# Autodesk Inventor assembly: UpperBody
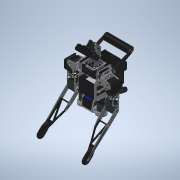
[picture p0: Inventor's stored thumbnail of the model, 180x180]
Saved by Autodesk Inventor 2020.4 (Build 244396000, 396)
## iProperties
Created: 2016-05-03
Part Number: UpperBody
Document SubType Name: Assembly
Designer: hiroaki
Mass: 2419.66 g
Surface Area: 8002.44 cm^2
Volume: 1435.02 cm^3
Density: 1.68615 g/cm^3
Author: hiroaki
## Documents named in this file (9)
- C:\Users\Masato\Documents\Inventor\CIT Brains_Inventor\OpenPlatform_ver3_0\UpperBody.iam
- C:\Users\Masato\Documents\Inventor\CIT Brains_Inventor\OpenPlatform_ver3_0\UpperBody\Trunk\Trunk.iam
- C:\Users\Masato\Documents\Inventor\CIT Brains_Inventor\OpenPlatform_ver3_0\UpperBody\Head\Head.iam
- C:\Users\Masato\Documents\Inventor\CIT Brains_Inventor\OpenPlatform_ver3_0\UpperBody\Arm\ForeArm.iam
- C:\Users\Masato\Documents\Inventor\CIT Brains_Inventor\OpenPlatform_ver3_0\UpperBody\Arm\Shoulder.iam
- C:\Users\Masato\Documents\Inventor\CIT Brains_Inventor\OpenPlatform_ver3_0\UpperBody\Arm\UpperArm.iam
- C:\Users\Masato\Documents\Inventor\CIT Brains_Inventor\OpenPlatform_ver3_0\UpperBody\Arm\SideBumper.ipt
- C:\Users\Masato\Documents\Inventor\CIT Brains_Inventor\OpenPlatform_ver3_0\Ready_Made\Screw\M2_6-6.ipt
- C:\Users\Masato\Documents\Inventor\CIT Brains_Inventor\OpenPlatform_ver3_0\Ready_Made\Screw\M2_6-8.ipt
## Components (54 placed, 8 different names)
1. Head:1 [sub-assembly] — 挿入:13, 角度:12, 挿入:82, 挿入:83, 挿入:84, 挿入:85
2. Trunk:1 [sub-assembly] — 挿入:13, 角度:12, 挿入:22, 挿入:23, 角度:22
3. ForeArm:1 [sub-assembly] — 角度:18, 挿入:21, 角度:19, 挿入:66, 挿入:67, 挿入:68, 挿入:69, 挿入:70, 挿入:71, 挿入:72, 挿入:73
4. UpperArm:1 [sub-assembly] — 挿入:21, 角度:19, メイト:4, 角度:20, メイト:5, 挿入:25
5. ForeArm:2 [sub-assembly] — 挿入:19, 角度:18, 挿入:74, 挿入:75, 挿入:76, 挿入:77, 挿入:78, 挿入:79, 挿入:80, 挿入:81
6. UpperArm:2 [sub-assembly] — 挿入:19, メイト:3, 角度:21, メイト:6, 挿入:24
7. SideBumper:1 — メイト:4, 角度:20, メイト:5
8. SideBumper:2 — メイト:3, 角度:21, メイト:6
9. Shoulder:1 [sub-assembly] — 挿入:22, 挿入:25, 角度:22, 角度:23, 挿入:42, 挿入:43, 挿入:44, 挿入:45, 挿入:46, 挿入:47, 挿入:48, 挿入:49, 挿入:50, 挿入:51, 挿入:52, 挿入:53
10. Shoulder:2 [sub-assembly] — 挿入:23, 挿入:24, 角度:23, 挿入:54, 挿入:55, 挿入:56, 挿入:57, 挿入:58, 挿入:59, 挿入:60, 挿入:61, 挿入:62, 挿入:63, 挿入:64, 挿入:65
11. M2_6-6:1 — 挿入:42
12. M2_6-6:2 — 挿入:43
13. M2_6-6:3 — 挿入:44
14. M2_6-6:4 — 挿入:45
15. M2_6-6:5 — 挿入:46
16. M2_6-6:6 — 挿入:47
17. M2_6-6:7 — 挿入:48
18. M2_6-6:8 — 挿入:49
19. M2_6-6:9 — 挿入:50
20. M2_6-6:10 — 挿入:51
21. M2_6-6:11 — 挿入:52
22. M2_6-6:12 — 挿入:53
23. M2_6-6:13 — 挿入:54
24. M2_6-6:14 — 挿入:55
25. M2_6-6:15 — 挿入:56
26. M2_6-6:16 — 挿入:57
27. M2_6-6:17 — 挿入:58
28. M2_6-6:18 — 挿入:59
29. M2_6-6:19 — 挿入:60
30. M2_6-6:20 — 挿入:61
31. M2_6-6:21 — 挿入:62
32. M2_6-6:22 — 挿入:63
33. M2_6-6:23 — 挿入:64
34. M2_6-6:24 — 挿入:65
35. M2_6-6:25 — 挿入:66
36. M2_6-6:26 — 挿入:67
37. M2_6-6:27 — 挿入:68
38. M2_6-6:28 — 挿入:69
39. M2_6-6:29 — 挿入:70
40. M2_6-6:30 — 挿入:71
41. M2_6-6:31 — 挿入:72
42. M2_6-6:32 — 挿入:73
43. M2_6-6:33 — 挿入:74
44. M2_6-6:34 — 挿入:75
45. M2_6-6:35 — 挿入:76
46. M2_6-6:36 — 挿入:77
47. M2_6-6:37 — 挿入:78
48. M2_6-6:38 — 挿入:79
49. M2_6-6:39 — 挿入:81
50. M2_6-6:40 — 挿入:80
51. M2_6-8:1 — 挿入:82
52. M2_6-8:2 — 挿入:83
53. M2_6-8:3 — 挿入:84
54. M2_6-8:4 — 挿入:85
## Relationships (62: Insert 51, Angle 7, Mate 4)
- 挿入:13 [Insert]: Head:1 ↔ Trunk:1
- 角度:12 [Angle] (0 deg): Head:1 ↔ Trunk:1
- 挿入:19 [Insert]: ForeArm:2 ↔ UpperArm:2
- 角度:18 [Angle] (0 deg): ForeArm:1 ↔ ForeArm:2
- 挿入:21 [Insert]: ForeArm:1 ↔ UpperArm:1
- 角度:19 [Angle] (45 deg): ForeArm:1 ↔ UpperArm:1
- メイト:3 [Mate]: UpperArm:2 ↔ SideBumper:2
- メイト:4 [Mate]: UpperArm:1 ↔ SideBumper:1
- 角度:20 [Angle] (0 deg): UpperArm:1 ↔ SideBumper:1
- メイト:5 [Mate]: UpperArm:1 ↔ SideBumper:1
- 角度:21 [Angle] (0 deg): UpperArm:2 ↔ SideBumper:2
- メイト:6 [Mate]: UpperArm:2 ↔ SideBumper:2
- 挿入:22 [Insert]: Trunk:1 ↔ Shoulder:1
- 挿入:23 [Insert]: Trunk:1 ↔ Shoulder:2
- 挿入:24 [Insert]: UpperArm:2 ↔ Shoulder:2
- 挿入:25 [Insert]: UpperArm:1 ↔ Shoulder:1
- 角度:22 [Angle] (0 deg): Trunk:1 ↔ Shoulder:1
- 角度:23 [Angle] (0 deg): Shoulder:1 ↔ Shoulder:2
- 挿入:42 [Insert]: Shoulder:1 ↔ M2_6-6:1
- 挿入:43 [Insert]: Shoulder:1 ↔ M2_6-6:2
- 挿入:44 [Insert]: Shoulder:1 ↔ M2_6-6:3
- 挿入:45 [Insert]: Shoulder:1 ↔ M2_6-6:4
- 挿入:46 [Insert]: Shoulder:1 ↔ M2_6-6:5
- 挿入:47 [Insert]: Shoulder:1 ↔ M2_6-6:6
- 挿入:48 [Insert]: Shoulder:1 ↔ M2_6-6:7
- 挿入:49 [Insert]: Shoulder:1 ↔ M2_6-6:8
- 挿入:50 [Insert]: Shoulder:1 ↔ M2_6-6:9
- 挿入:51 [Insert]: Shoulder:1 ↔ M2_6-6:10
- 挿入:52 [Insert]: Shoulder:1 ↔ M2_6-6:11
- 挿入:53 [Insert]: Shoulder:1 ↔ M2_6-6:12
- 挿入:54 [Insert]: Shoulder:2 ↔ M2_6-6:13
- 挿入:55 [Insert]: Shoulder:2 ↔ M2_6-6:14
- 挿入:56 [Insert]: Shoulder:2 ↔ M2_6-6:15
- 挿入:57 [Insert]: Shoulder:2 ↔ M2_6-6:16
- 挿入:58 [Insert]: Shoulder:2 ↔ M2_6-6:17
- 挿入:59 [Insert]: Shoulder:2 ↔ M2_6-6:18
- 挿入:60 [Insert]: Shoulder:2 ↔ M2_6-6:19
- 挿入:61 [Insert]: Shoulder:2 ↔ M2_6-6:20
- 挿入:62 [Insert]: Shoulder:2 ↔ M2_6-6:21
- 挿入:63 [Insert]: Shoulder:2 ↔ M2_6-6:22
- 挿入:64 [Insert]: Shoulder:2 ↔ M2_6-6:23
- 挿入:65 [Insert]: Shoulder:2 ↔ M2_6-6:24
- 挿入:66 [Insert]: ForeArm:1 ↔ M2_6-6:25
- 挿入:67 [Insert]: ForeArm:1 ↔ M2_6-6:26
- 挿入:68 [Insert]: ForeArm:1 ↔ M2_6-6:27
- 挿入:69 [Insert]: ForeArm:1 ↔ M2_6-6:28
- 挿入:70 [Insert]: ForeArm:1 ↔ M2_6-6:29
- 挿入:71 [Insert]: ForeArm:1 ↔ M2_6-6:30
- 挿入:72 [Insert]: ForeArm:1 ↔ M2_6-6:31
- 挿入:73 [Insert]: ForeArm:1 ↔ M2_6-6:32
- 挿入:74 [Insert]: ForeArm:2 ↔ M2_6-6:33
- 挿入:75 [Insert]: ForeArm:2 ↔ M2_6-6:34
- 挿入:76 [Insert]: ForeArm:2 ↔ M2_6-6:35
- 挿入:77 [Insert]: ForeArm:2 ↔ M2_6-6:36
- 挿入:78 [Insert]: ForeArm:2 ↔ M2_6-6:37
- 挿入:79 [Insert]: ForeArm:2 ↔ M2_6-6:38
- 挿入:80 [Insert]: ForeArm:2 ↔ M2_6-6:40
- 挿入:81 [Insert]: ForeArm:2 ↔ M2_6-6:39
- 挿入:82 [Insert]: Head:1 ↔ M2_6-8:1
- 挿入:83 [Insert]: Head:1 ↔ M2_6-8:2
- 挿入:84 [Insert]: Head:1 ↔ M2_6-8:3
- 挿入:85 [Insert]: Head:1 ↔ M2_6-8:4
